# Autodesk Inventor assembly: SLHSSW10
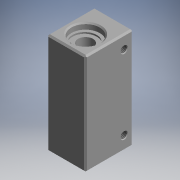
[picture p0: Inventor's stored thumbnail of the model, 180x180]
Saved by Autodesk Inventor 2017.3 (Build 213256000, 256)
## iProperties
Category: PARTsolutions
Company: MISUMI
Part Number: SLHSSW10
Catalog Web Link: www.cadenas.de
Description: LHSSW, LHSSWF, SLHSSW, SLHSSWF-Linear Bushing Pillow Blocks - Standard Tall Blocks, Double
Vendor: MISUMI
Document SubType Name: Assembly
Designer: partserver
Manufacturer: MISUMI
Mass: 47.3945 g
Surface Area: 202.244 cm^2
Volume: 47.3945 cm^3
Density: 1 g/cm^3
Title: SLHSSW10
Author: Cadenas PARTsolutions
Comments: Linear Bushing Pillow Blocks - Standard Tall Blocks, Double
PSOL_IDENT_0: {$CADENAS_DATA\23d-libs\misumi\metric\04_linear_bushings\lhssw_asmtab.prj},203 {VTYP=3D},{STYP=ASSTA
PSOL_IDENT_1: B},{NB=SLHSSW10},{LINA=SLHSSW10},{NN=LHSSW, LHSSWF, SLHSSW, SLHSSWF},{DATE=06.10.2021 02:05:36},{GEO
PSOL_IDENT_2: MDATE=06.10.2021 02:04:59},{VERSION=},{LINEID=90},{WBVAR=LB,GREASE},{WBNUMERIC=}  {NB=SLHSSW10},{LIN
PSOL_IDENT_3: A=SLHSSW10},{KT=DUMMY},{PN=SLHSSW10},{TYPE=SLHSSW},{LB=SLMU},{LBALG= 'LMU', 'LMU', 'LMUF', 'LMUF', '
PSOL_IDENT_4: SLMU', 'SLMU', 'SLMUS', 'SLMUS' },{GREASE=},{DDRR=10},{D=19},{RRTS=S},{RRNO=19},{S=4.0},{RRW=1.15},{
PSOL_IDENT_5: RRD=20.0},{RRC=0.8},{L=68},{L1=36},{L2=50},{HH=19},{W=26},{H=32},{LL=6},{M1=M6 (9.5)},{M13D=6},{M2=M
PSOL_IDENT_6: 5 (20)},{M23D=5},{C1=(1)},{DD1TT=8x6 (for M4 Bolt)},{DD1=8.0},{TT=6.0},{PPATH=lhssw/lhssw_asmtpl.prj
PSOL_IDENT_7: }
NB: SLHSSW10
NN: LHSSW, LHSSWF, SLHSSW, SLHSSWF
NT: Linear Bushing Pillow Blocks - Standard Tall Blocks, Double
NBSYN: $PN.
LINA: SLHSSW10
CATALOG: Misumi
PN: SLHSSW10
LB: SLMU
GREASE: Not Provided
DDRR: 10
D: 19
S: 4
L: 68
L1: 36
L2: 50
HH: 19
W: 26
H: 32
LL: 6
M1: M6 (9.5)
M2: M5 (20)
C1: (1)
DD1TT: 8x6 (for M4 Bolt)
SUPPLIER: MISUMI
ARTICLENO: SLHSSW10
BOMINFO: SLHSSW10
CREATOR: CADENAS GmbH
## Documents named in this file (4)
- e:\temp\worker_21\temp\exporttempdir_2444_229_n8Yr2\format_0\SLHSSW10.iam
- e:\temp\worker_21\temp\exporttempdir_2444_229_n8Yr2\format_0\SLHSSW10_b.ipt
- e:\temp\worker_21\temp\exporttempdir_2444_229_n8Yr2\format_0\BUSHING_REFERENCE_DATA_FOR_LHSSW10.ipt
- e:\temp\worker_21\temp\exporttempdir_2444_229_n8Yr2\format_0\LH-RRING-C-INT-S-19.ipt
## Components (4 placed, 3 different names)
1. SLHSSW10_b:1 — to_bushings_XY@1 <-> to_housing_XY@2, to_bushings_Z@1 <-> to_housing_Z@2, to_bushings_YZ@1 <-> to_housing_YZ@2, to_rring_l_XY@1 <-> rr_XY@3, to_rring_l_Z@1 <-> rr_Z@3, to_rring_l_YZ@1 <-> rr_YZ@3, to_rring_r_XY@1 <-> rr_XY@4, to_rring_r_Z@1 <-> rr_Z@4, to_rring_r_YZ@1 <-> rr_YZ@4
2. BUSHING_REFERENCE_DATA_FOR_LHSSW10:1 — to_bushings_XY@1 <-> to_housing_XY@2, to_bushings_Z@1 <-> to_housing_Z@2, to_bushings_YZ@1 <-> to_housing_YZ@2
3. LH-RRING-C-INT-S-19:1 — to_rring_l_XY@1 <-> rr_XY@3, to_rring_l_Z@1 <-> rr_Z@3, to_rring_l_YZ@1 <-> rr_YZ@3
4. LH-RRING-C-INT-S-19:2 — to_rring_r_XY@1 <-> rr_XY@4, to_rring_r_Z@1 <-> rr_Z@4, to_rring_r_YZ@1 <-> rr_YZ@4
## Relationships (9: Mate 6, Angle 3)
- to_bushings_XY@1 <-> to_housing_XY@2 [Mate]: SLHSSW10_b:1 ↔ BUSHING_REFERENCE_DATA_FOR_LHSSW10:1
- to_bushings_Z@1 <-> to_housing_Z@2 [Mate]: SLHSSW10_b:1 ↔ BUSHING_REFERENCE_DATA_FOR_LHSSW10:1
- to_bushings_YZ@1 <-> to_housing_YZ@2 [Angle] (0 deg): SLHSSW10_b:1 ↔ BUSHING_REFERENCE_DATA_FOR_LHSSW10:1
- to_rring_l_XY@1 <-> rr_XY@3 [Mate]: SLHSSW10_b:1 ↔ LH-RRING-C-INT-S-19:1
- to_rring_l_Z@1 <-> rr_Z@3 [Mate]: SLHSSW10_b:1 ↔ LH-RRING-C-INT-S-19:1
- to_rring_l_YZ@1 <-> rr_YZ@3 [Angle] (0 deg): SLHSSW10_b:1 ↔ LH-RRING-C-INT-S-19:1
- to_rring_r_XY@1 <-> rr_XY@4 [Mate]: SLHSSW10_b:1 ↔ LH-RRING-C-INT-S-19:2
- to_rring_r_Z@1 <-> rr_Z@4 [Mate]: SLHSSW10_b:1 ↔ LH-RRING-C-INT-S-19:2
- to_rring_r_YZ@1 <-> rr_YZ@4 [Angle] (0 deg): SLHSSW10_b:1 ↔ LH-RRING-C-INT-S-19:2
